# Autodesk Inventor assembly: GPS Module
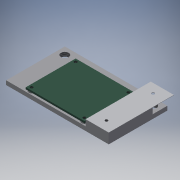
[picture p0: Inventor's stored thumbnail of the model, 180x180]
Saved by Autodesk Inventor 2019 (Build 230136000, 136)
## iProperties
Created: 2020-08-03
Part Number: GPS Module
Document SubType Name: Assembly
Designer: james
Author: james
## Documents named in this file (4)
- F:\JimsRobot\FIRSTRobots\Design\Library\Jims\GPS Module.iam
- F:\JimsRobot\FIRSTRobots\Design\Library\Jims\SF GPS.ipt
- F:\JimsRobot\FIRSTRobots\Design\Library\Sparkfun\Molex Flexible GNSS Antenna.ipt
- F:\JimsRobot\FIRSTRobots\Design\Library\Sparkfun\SparkFun GPS-RTK Dead Reckoning Breakout.ipt
## Components (3 placed, 3 different names)
1. SF GPS:1 — Mate:1, Mate:2, Mate:3, Mate:4, Mate:5
2. Molex Flexible GNSS Antenna:1 — Mate:3, Mate:4
3. SparkFun GPS-RTK Dead Reckoning Breakout:1 — Mate:1, Mate:2, Mate:5
## Relationships (5: Mate 5)
- Mate:1: SF GPS:1 ↔ SparkFun GPS-RTK Dead Reckoning Breakout:1
- Mate:2: SF GPS:1 ↔ SparkFun GPS-RTK Dead Reckoning Breakout:1
- Mate:3: SF GPS:1 ↔ Molex Flexible GNSS Antenna:1
- Mate:4: SF GPS:1 ↔ Molex Flexible GNSS Antenna:1
- Mate:5: SF GPS:1 ↔ SparkFun GPS-RTK Dead Reckoning Breakout:1
